# Autodesk Inventor assembly: 16-3
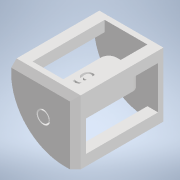
[picture p0: Inventor's stored thumbnail of the model, 180x180]
Saved by Autodesk Inventor 2022 (Build 260153000, 153)
## iProperties
Created: 2021-09-25
Part Number: 16-3
Document SubType Name: Assembly
Designer: 서울공업고등학교
Author: 서울공업고등학교
## Documents named in this file (3)
- C:\Users\서울공업고등학교\Downloads\3dPrinter-main\_9_25\16번\16-3.iam
- C:\Users\서울공업고등학교\Downloads\3dPrinter-main\_9_25\16번\16-1.ipt
- C:\Users\서울공업고등학교\Downloads\3dPrinter-main\_9_25\16번\16-2.ipt
## Components (2 placed, 2 different names)
1. 16-1:1 — 메이트:1, 메이트:2
2. 16-2:1 — 메이트:1, 메이트:2
## Relationships (2: Mate 2)
- 메이트:1 [Mate]: 16-1:1 ↔ 16-2:1
- 메이트:2 [Mate] (0.5 mm): 16-1:1 ↔ 16-2:1
